# Autodesk Inventor assembly: valve-solenoid
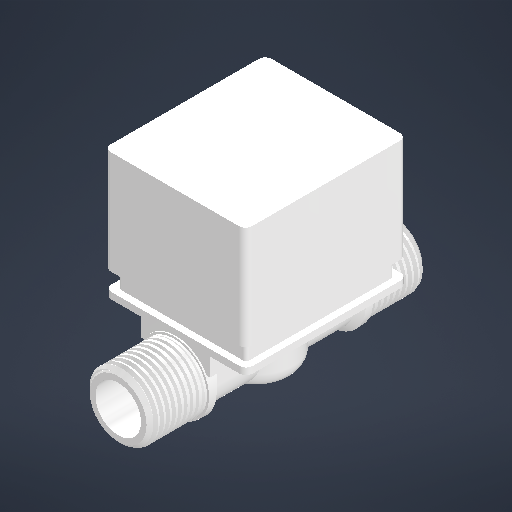
[picture p0: Inventor's stored thumbnail of the model, 512x512]
Saved by Autodesk Inventor 2025.2 (Build 292293000, 293)
## iProperties
Created: 2026-01-02
Part Number: valve-solenoid
Document SubType Name: Assembly
Designer: sam
Author: sam
## iProperties of the stored document solenoid-valve.ipt
Created: 2021-07-30
Part Number: solenoid-valve
Material: ABS Plastic
Description: STEP AP203
Document SubType Name: Modeling
Designer: sam
Density: 1.06 g/cm^3
Appearance: Smooth - White
Sending System: SolidWorks 2014
Preprocessor: SwSTEP 2.0
Title: solenoid valwe.STEP
Revision Number: ANY
## Documents named in this file (4)
- **G:\projects\primary\regulated-irrigation-system\model\asm\electronic-components\valve-solenoid\valve-solenoid.iam*LocalDocs*xAaaaqtcaAaaaaaaaAaaaa5fpGh*solenoid-valve.ipt
- G:\projects\primary\regulated-irrigation-system\model\asm\electronic-components\valve-solenoid\valve-solenoid.iam
- G:\projects\primary\regulated-irrigation-system\model\asm\electronic-components\valve-solenoid\encloser_valve-solenoid.ipt
- G:\projects\primary\regulated-irrigation-system\model\asm\electronic-components\valve-solenoid\solenoid-valve.STEP
## Components (2 placed, 2 different names)
1. solenoid-valve:1 — Mate:1, Mate:2, Mate:3
2. encloser_valve-solenoid:1 — Mate:1, Mate:2, Mate:3
## Relationships (3: Mate 3)
- Mate:1 (0.4 mm): solenoid-valve:1 ↔ encloser_valve-solenoid:1
- Mate:2 (0.2 mm): solenoid-valve:1 ↔ encloser_valve-solenoid:1
- Mate:3 (0.2 mm): solenoid-valve:1 ↔ encloser_valve-solenoid:1
